# Autodesk Inventor assembly: Anglerfish_VCM_v2
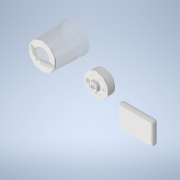
[picture p0: Inventor's stored thumbnail of the model, 180x180]
Saved by Autodesk Inventor 2022 (Build 260153000, 153)
## iProperties
Created: 2022-04-02
Part Number: Anglerfish_VCM_v2
Document SubType Name: Assembly
Designer: Prakash Lab
Author: Prakash Lab
## Documents named in this file (11)
- C:\Users\diederichbenedict\Documents\GitHub\Matchboxscope\INVENTOR\Anglerfish_VCM_v2.iam
- C:\Users\diederichbenedict\Documents\GitHub\Matchboxscope\INVENTOR\00_ESP3-CAM.iam
- C:\Users\diederichbenedict\Documents\GitHub\Matchboxscope\INVENTOR\00_Powerbank.ipt
- C:\Users\diederichbenedict\Documents\Inventor\Content Center Files\R2022\de-DE\DIN 912\DIN 912 - M3 x 0.5 x 25 x 18.ipt
- C:\Users\diederichbenedict\Documents\GitHub\Matchboxscope\INVENTOR\00_bonne_maman_jar.ipt
- C:\Users\diederichbenedict\Documents\GitHub\Matchboxscope\INVENTOR\Anglerfish_Jar_Adapterplate_v1.ipt
- C:\Users\diederichbenedict\Documents\GitHub\Matchboxscope\INVENTOR\Anglerfish_bottom_v0.ipt
- C:\Users\diederichbenedict\Documents\GitHub\Matchboxscope\INVENTOR\Anglerfish_middle2_m12VCMLens_v2.ipt
- C:\Users\diederichbenedict\Documents\GitHub\Matchboxscope\INVENTOR\00_CCTV_M12_VCM.ipt
- C:\Users\diederichbenedict\Documents\GitHub\Matchboxscope\INVENTOR\Matchboxscope_M12_Lensadapter_v0.ipt
- C:\Users\diederichbenedict\Documents\GitHub\Matchboxscope\INVENTOR\Anglerfish_Lightplate.ipt
## Components (12 placed, 10 different names)
1. Anglerfish_middle2_m12VCMLens_v2:1 — Insert:1, Angle:1, Mate:5, Einfügen:2
2. Anglerfish_bottom_v0:1 — Mate:1, Mate:2, Mate:3, Mate:4, Flush:1, Mate:5, Passend:6
3. 00_ESP3-CAM:1 [sub-assembly] — Mate:4, Flush:1, Insert:1
4. 00_Powerbank:1
5. 00_bonne_maman_jar:1 — Winkel:2, Fluchtend:2, Fluchtend:3
6. DIN 912 - ersetzt durch DIN EN ISO 4762 M3 x 25:5
7. DIN 912 - ersetzt durch DIN EN ISO 4762 M3 x 25:7
8. DIN 912 - ersetzt durch DIN EN ISO 4762 M3 x 25:8
9. 00_CCTV_M12_VCM:1 — Einfügen:2, Einfügen:3
10. Matchboxscope_M12_Lensadapter_v0:1 — Einfügen:3
11. Anglerfish_Jar_Adapterplate_v1:1 — Passend:6
12. Anglerfish_Lightplate:1 — Fluchtend:2, Fluchtend:3
## Relationships (14: Mate 6, Flush 3, Insert 3, Angle 2)
- Mate:1: Anglerfish_bottom_v0:1
- Mate:2: Anglerfish_bottom_v0:1
- Mate:3: Anglerfish_bottom_v0:1
- Mate:4: Anglerfish_bottom_v0:1 ↔ 00_ESP3-CAM:1
- Flush:1: Anglerfish_bottom_v0:1 ↔ 00_ESP3-CAM:1
- Insert:1: Anglerfish_middle2_m12VCMLens_v2:1 ↔ 00_ESP3-CAM:1
- Angle:1 (0 deg): Anglerfish_middle2_m12VCMLens_v2:1
- Mate:5: Anglerfish_middle2_m12VCMLens_v2:1 ↔ Anglerfish_bottom_v0:1
- Winkel:2 [Angle] (0 deg): 00_bonne_maman_jar:1
- Passend:6 [Mate]: Anglerfish_bottom_v0:1 ↔ Anglerfish_Jar_Adapterplate_v1:1
- Einfügen:2 [Insert]: Anglerfish_middle2_m12VCMLens_v2:1 ↔ 00_CCTV_M12_VCM:1
- Einfügen:3 [Insert] (-2 mm): 00_CCTV_M12_VCM:1 ↔ Matchboxscope_M12_Lensadapter_v0:1
- Fluchtend:2 [Flush]: 00_bonne_maman_jar:1 ↔ Anglerfish_Lightplate:1
- Fluchtend:3 [Flush]: 00_bonne_maman_jar:1 ↔ Anglerfish_Lightplate:1
